# Autodesk Inventor assembly: Front Hub Carrier R new
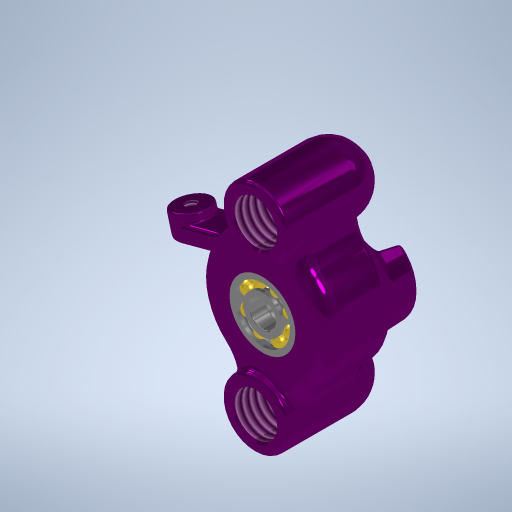
[picture p0: Inventor's stored thumbnail of the model, 512x512]
Saved by Autodesk Inventor 2023 (Build 270158000, 158)
## iProperties
Created: 2023-03-24
Part Number: Front Hub Carrier R new
Document SubType Name: Assembly
Designer: CASPER
Author: CASPER
## Documents named in this file (3)
- C:\Users\CASPER\Desktop\HUDSON süspansiyon\Front Hub Carrier R new.iam
- C:\Users\CASPER\Desktop\HUDSON süspansiyon\Front Hub Carrier R.ipt
- C:\Users\CASPER\Desktop\Rulman(fixed)\Assemblybearing.iam
## Components (3 placed, 2 different names)
1. Front Hub Carrier R:1 — Mate:1, Mate:2, Mate:3, Mate:4, Mate:5, Mate:6
2. Assemblybearing:1 [sub-assembly] — Mate:1, Mate:2, Mate:3, Mate:4
3. Assemblybearing:2 [sub-assembly] — Mate:5, Mate:6
## Relationships (6: Mate 6)
- Mate:1: Front Hub Carrier R:1 ↔ Assemblybearing:1
- Mate:2: Front Hub Carrier R:1 ↔ Assemblybearing:1
- Mate:3: Front Hub Carrier R:1 ↔ Assemblybearing:1
- Mate:4: Front Hub Carrier R:1 ↔ Assemblybearing:1
- Mate:5: Front Hub Carrier R:1 ↔ Assemblybearing:2
- Mate:6: Front Hub Carrier R:1 ↔ Assemblybearing:2
